# Autodesk Inventor assembly: Gehause_Fitting
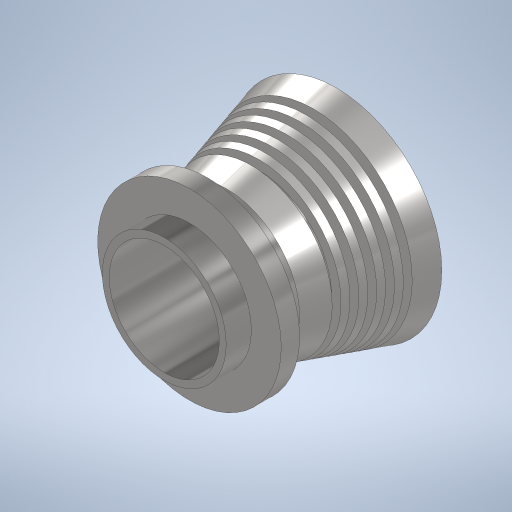
[picture p0: Inventor's stored thumbnail of the model, 512x512]
Saved by Autodesk Inventor 2024 (Build 280153000, 153)
## iProperties
Created: 2024-03-08
Part Number: Gehause_Fitting
Document SubType Name: Assembly
Designer: ffogue
Author: ffogue
## Documents named in this file (3)
- C:\Users\ffogue\OneDrive - MuM - OM\Dokumente\Inventor\Stermotor\Gehause_Fitting.iam
- C:\Users\ffogue\OneDrive - MuM - OM\Dokumente\Inventor\Stermotor\gehäuse_winkel_bohrung.ipt
- C:\Users\ffogue\OneDrive - MuM - OM\Dokumente\Inventor\Stermotor\fitting.ipt
## Components (2 placed, 2 different names)
1. gehäuse_winkel_bohrung:1 — Passend:1
2. fitting:1 — Passend:1
## Relationships (1: Mate 1)
- Passend:1 [Mate]: gehäuse_winkel_bohrung:1 ↔ fitting:1
